# Autodesk Inventor assembly: Chasis_03
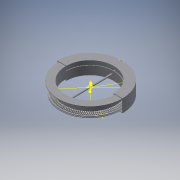
[picture p0: Inventor's stored thumbnail of the model, 180x180]
Saved by Autodesk Inventor 2017 (Build 210142000, 142)
## iProperties
Created: 2017-01-10
Part Number: Chasis_03
Document SubType Name: Assembly
Designer: David Kopala
Author: David Kopala
## Documents named in this file (6)
- Z:\Documents\Drone\Drone\3D Models\Project\Chasis_03\Chasis_03.iam
- Z:\Documents\Drone\Drone\3D Models\Project\Chasis_03\Outer_Shell.ipt
- Z:\Documents\Drone\Drone\3D Models\Project\Chasis_03\BevelSystem.iam
- Z:\Documents\Drone\Drone\3D Models\Project\Chasis_03\MotorMount.iam
- Z:\Documents\Drone\Drone\3D Models\Project\Chasis_03\Layer2_Ref.ipt
- Z:\Documents\Drone\Drone\3D Models\Project\Chasis_03\Spur_Reference\Design Accelerator\Spur Gear11.ipt
## Components (5 placed, 5 different names)
1. Outer_Shell:1 — Insert:2
2. BevelSystem:1 [sub-assembly] — Insert:3
3. MotorMount:1 [sub-assembly]
4. Layer2_Ref:1 — Insert:2, Insert:3, Insert:4
5. Spur Gear1:1 — Insert:4
## Relationships (3: Insert 3)
- Insert:2 (1.5875 mm): Outer_Shell:1 ↔ Layer2_Ref:1
- Insert:3 (1.5875 mm): BevelSystem:1 ↔ Layer2_Ref:1
- Insert:4: Layer2_Ref:1 ↔ Spur Gear1:1
